# Autodesk Inventor assembly: Synchronous Belts Transmission
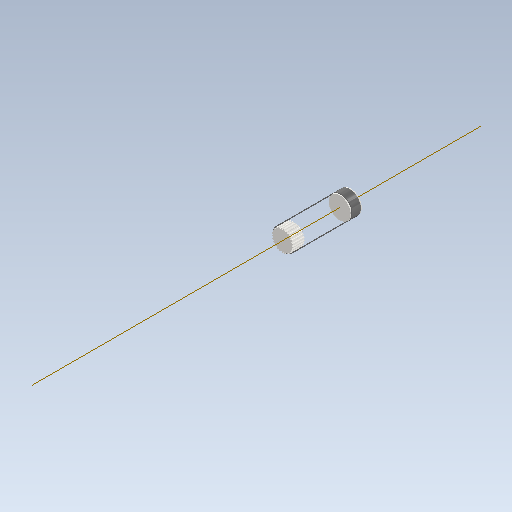
[picture p0: Inventor's stored thumbnail of the model, 512x512]
Saved by Autodesk Inventor 2020 (Build 240168000, 168)
## iProperties
ClientObjectVersion: 1
Created: 2022-07-06
Part Number: Synchronous Belts Transmission
Document SubType Name: Assembly
Designer: karimi2
Author: karimi2
## Documents named in this file (4)
- C:\Users\karimi2\Documents\PROJECT\src\Assembly1\Design Accelerator\Synchronous Belts Transmission1.iam
- C:\Users\karimi2\Documents\PROJECT\src\Assembly1\Design Accelerator\Synchronous Belt1.ipt
- C:\Users\karimi2\Documents\PROJECT\src\Assembly1\Design Accelerator\Synchronous Pulley11.ipt
- C:\Users\karimi2\Documents\PROJECT\src\Assembly1\Design Accelerator\Synchronous Pulley21.ipt
## Components (3 placed, 3 different names)
1. Synchronous Belt:1 — Flush:1, Mate:1, Mate:2, Flush:2, Mate:3, Mate:4
2. Synchronous Pulley1:1 — Flush:1, Mate:1, Mate:2, Rotation:1
3. Synchronous Pulley2:1 — Flush:2, Mate:3, Rotation:1, Mate:4
## Relationships (7: Mate 4, Flush 2, RelateRotation 1)
- Flush:1: Synchronous Belt:1 ↔ Synchronous Pulley1:1
- Mate:1: Synchronous Belt:1 ↔ Synchronous Pulley1:1
- Mate:2: Synchronous Belt:1 ↔ Synchronous Pulley1:1
- Flush:2: Synchronous Belt:1 ↔ Synchronous Pulley2:1
- Mate:3: Synchronous Belt:1 ↔ Synchronous Pulley2:1
- Rotation:1 [RelateRotation] (1 ul): Synchronous Pulley1:1 ↔ Synchronous Pulley2:1
- Mate:4: Synchronous Belt:1 ↔ Synchronous Pulley2:1
